# Autodesk Inventor assembly: NewComplet
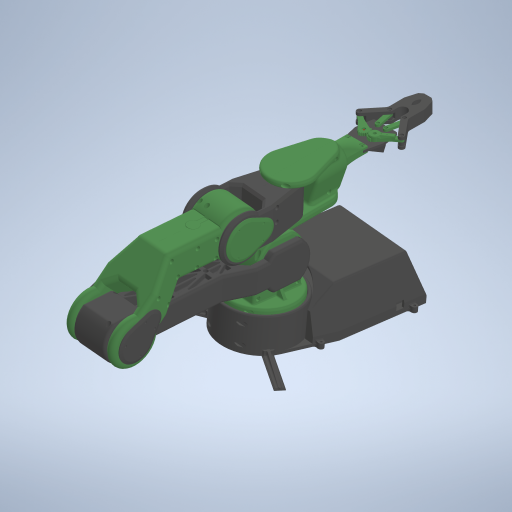
[picture p0: Inventor's stored thumbnail of the model, 512x512]
Saved by Autodesk Inventor 2023 (Build 270158000, 158)
## iProperties
Created: 2024-07-23
Part Number: NewComplet
Document SubType Name: Assembly
Designer: Swoby
Author: Swoby
## Documents named in this file (5)
- C:\Users\Swoby\OneDrive\Plocha\DUM-E\V0.3\NewComplet.iam
- C:\Users\Swoby\OneDrive\Plocha\DUM-E\V0.3\NewGripper\Gripper.iam
- C:\Users\Swoby\OneDrive\Plocha\DUM-E\V0.3\NewWirst\Wrist.iam
- C:\Users\Swoby\OneDrive\Plocha\DUM-E\V0.3\NewArm\Arm.iam
- C:\Users\Swoby\OneDrive\Plocha\DUM-E\V0.3\NewBase\Base.iam
## Components (4 placed, 4 different names)
1. Gripper:1 [sub-assembly] — Mate:1, Mate:2
2. Wrist:1 [sub-assembly] — Mate:1, Mate:2, Mate:3, Mate:4
3. Arm:1 [sub-assembly] — Mate:3, Mate:4, Mate:5, Mate:6
4. Base:1 [sub-assembly] — Mate:5, Mate:6
## Relationships (6: Mate 6)
- Mate:1 (0.5 mm): Gripper:1 ↔ Wrist:1
- Mate:2: Gripper:1 ↔ Wrist:1
- Mate:3 (0.5 mm): Wrist:1 ↔ Arm:1
- Mate:4: Wrist:1 ↔ Arm:1
- Mate:5: Arm:1 ↔ Base:1
- Mate:6 (1 mm): Arm:1 ↔ Base:1
